# Autodesk Inventor assembly: アームアセンブリ
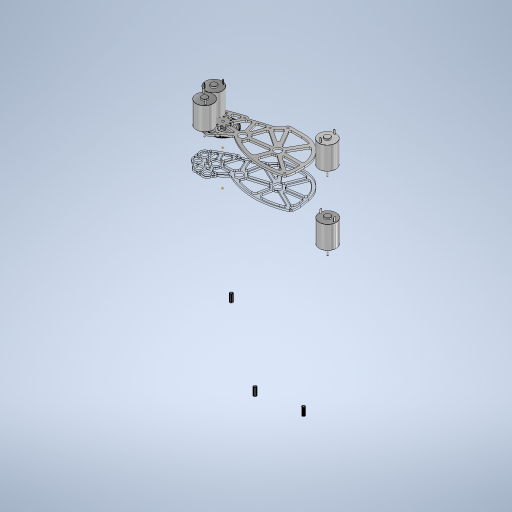
[picture p0: Inventor's stored thumbnail of the model, 512x512]
Saved by Autodesk Inventor 2023 (Build 270158000, 158)
## iProperties
Created: 2022-03-06
Part Number: アームアセンブリ
Document SubType Name: Assembly
Designer: acps
Author: acps
## Documents named in this file (6)
- C:\Users\acps\Documents\srdc\srdc_ksh\アーム\アームアセンブリ.iam
- C:\Users\acps\Documents\srdc\srdc_ksh\アーム\ギア\初段_多段ギア.iam
- C:\Users\acps\Documents\srdc\srdc_ksh\モータ\M-RS-380.ipt
- C:\Users\acps\Documents\srdc\srdc_ksh\アーム\ギアマウント.ipt
- C:\Users\acps\Documents\srdc\srdc_ksh\アーム\ギア\ぴにょん.ipt
- C:\Users\acps\Documents\srdc\srdc_ksh\アーム\ギアマウントポリカ.ipt
## Components (11 placed, 5 different names)
1. 初段_多段ギア:1 [sub-assembly] — Mate:2
2. M-RS-380:1
3. M-RS-380:2 — Mate:3, Insert:2
4. M-RS-380:3
5. M-RS-380:4 — Mate:1, Insert:1, Mate:4
6. ギアマウント:1 — Mate:1, Mate:2, Insert:1, Mate:3, Insert:2, Mate:5
7. ぴにょん:1 — Mate:4
8. ぴにょん:2
9. ぴにょん:3
10. ぴにょん:4
11. ギアマウントポリカ:1 — Mate:5
## Relationships (7: Mate 5, Insert 2)
- Mate:1: M-RS-380:4 ↔ ギアマウント:1
- Mate:2: 初段_多段ギア:1 ↔ ギアマウント:1
- Insert:1: M-RS-380:4 ↔ ギアマウント:1
- Mate:3: M-RS-380:2 ↔ ギアマウント:1
- Insert:2: M-RS-380:2 ↔ ギアマウント:1
- Mate:4: M-RS-380:4 ↔ ぴにょん:1
- Mate:5: ギアマウント:1 ↔ ギアマウントポリカ:1
